# Autodesk Inventor assembly: cnc_assembly_wo_z
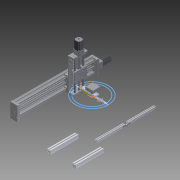
[picture p0: Inventor's stored thumbnail of the model, 180x180]
Saved by Autodesk Inventor 2011 (Build 150239000, 239)
## iProperties
Created: 2012-06-14
Part Number: cnc_assembly_wo_z
Document SubType Name: Assembly
Designer: labuser
Author: labuser
## Documents named in this file (7)
- C:\Users\labuser\Desktop\cnc_cad\cnc_assembly_wo_z.iam
- C:\Users\labuser\Desktop\cnc_cad\New XZ_Combo Master.iam
- C:\Users\labuser\Desktop\cnc_cad\nema_23.ipt
- C:\Users\labuser\Desktop\cnc_cad\head_assembly.iam
- C:\Users\labuser\Documents\GitHub\kinematic_mount\magnet_chuck_redesign\new_assembly.iam
- C:\Users\labuser\Desktop\cnc_cad\8020-40-4040-Lite.ipt
- C:\Users\labuser\Desktop\cnc_cad\8020-25-2525.ipt
## Components (9 placed, 6 different names)
1. New XZ_Combo Master:1 [sub-assembly] — Mate:1, Mate:3
2. nema_23:1 — Mate:3
3. nema_23:3 — Mate:1
4. head_assembly:1 [sub-assembly]
5. new_assembly:1 [sub-assembly] — Mate:16, Mate:17, Mate:18, Mate:19
6. 8020-40-4040-Lite:1
7. 8020-40-4040-Lite:2
8. 8020-25-2525:1 — Mate:16, Mate:17
9. 8020-25-2525:2 — Mate:18, Mate:19
## Relationships (6: Mate 6)
- Mate:1: New XZ_Combo Master:1 ↔ nema_23:3
- Mate:3: New XZ_Combo Master:1 ↔ nema_23:1
- Mate:16: new_assembly:1 ↔ 8020-25-2525:1
- Mate:17: new_assembly:1 ↔ 8020-25-2525:1
- Mate:18: new_assembly:1 ↔ 8020-25-2525:2
- Mate:19: new_assembly:1 ↔ 8020-25-2525:2
